# Autodesk Inventor assembly: Truss1
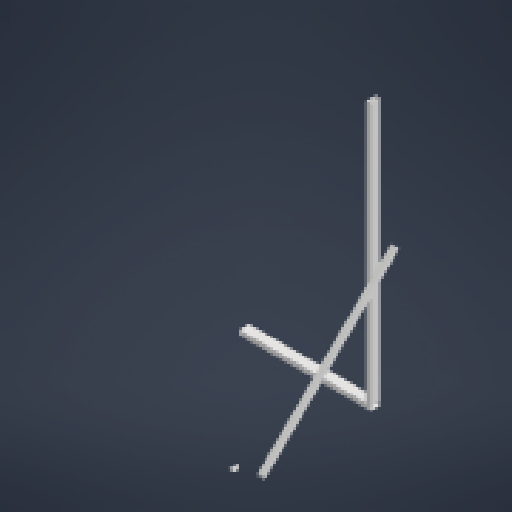
[picture p0: Inventor's stored thumbnail of the model, 512x512]
Saved by Autodesk Inventor 2023 (Build 270158000, 158)
## iProperties
Created: 2023-01-18
Part Number: Truss1
Document SubType Name: Assembly
Designer: Terrence
Author: Terrence
## Documents named in this file (5)
- C:\Users\Terrence\Documents\FRC Long\Truss\Truss1.iam
- C:\Users\Terrence\Documents\FRC Long\Truss\Solid1.ipt
- C:\Users\Terrence\Documents\FRC Long\Truss\Solid3.ipt
- C:\Users\Terrence\Documents\FRC Long\Truss\Solid6.ipt
- C:\Users\Terrence\Documents\FRC Long\Truss\Solid7.ipt
## Components (7 placed, 4 different names)
1. Solid1:1 — Mate:1, Flush:1, Flush:2, Insert:1, Insert:2
2. Solid3:1 — Mate:1, Flush:1, Flush:2, Flush:3, Mate:2, Flush:4
3. Solid6:1 — Insert:1, Insert:2, Insert:5, Insert:6
4. Solid7:1 — Insert:5, Insert:6
5. Solid1:2 — Flush:3, Mate:2, Flush:4, Insert:3, Insert:4
6. Solid6:2 — Insert:3, Insert:4, Insert:7, Insert:8
7. Solid7:3 — Insert:7, Insert:8
## Relationships (14: Insert 8, Flush 4, Mate 2)
- Mate:1: Solid1:1 ↔ Solid3:1
- Flush:1: Solid1:1 ↔ Solid3:1
- Flush:2: Solid1:1 ↔ Solid3:1
- Insert:1: Solid1:1 ↔ Solid6:1
- Insert:2: Solid1:1 ↔ Solid6:1
- Flush:3: Solid3:1 ↔ Solid1:2
- Mate:2: Solid3:1 ↔ Solid1:2
- Flush:4: Solid3:1 ↔ Solid1:2
- Insert:3: Solid1:2 ↔ Solid6:2
- Insert:4: Solid1:2 ↔ Solid6:2
- Insert:5: Solid6:1 ↔ Solid7:1
- Insert:6: Solid6:1 ↔ Solid7:1
- Insert:7: Solid6:2 ↔ Solid7:3
- Insert:8: Solid6:2 ↔ Solid7:3
